# Autodesk Inventor assembly: TTB Constant Force Spring Mount
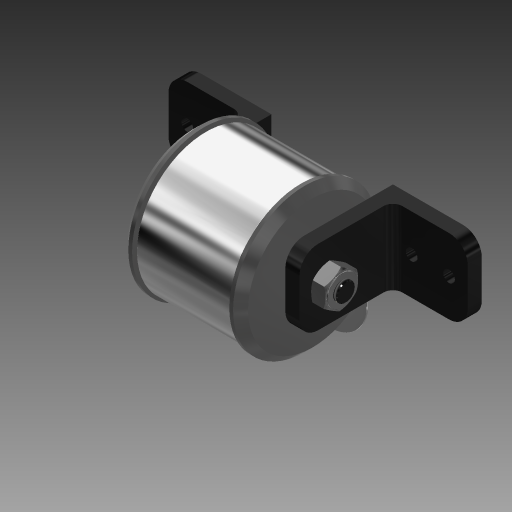
[picture p0: Inventor's stored thumbnail of the model, 512x512]
Saved by Autodesk Inventor 2023 (Build 270158000, 158)
## iProperties
Created: 2023-01-02
Part Number: TTB Constant Force Spring Mount
Document SubType Name: Assembly
Designer: Max Boord
Mass: 227.424 g
Surface Area: 355.542 cm^2
Volume: 75.7539 cm^3
Density: 3.00214 g/cm^3
Author: Max Boord
## iProperties of the stored document MemberDocs/xLcoxz3ngAkn1iylbNymdpbul3h
Created: 2023-01-02
Part Number: TTB Constant Force Spring Mount
Document SubType Name: Assembly
Designer: Max Boord
Mass: 227.424 g
Surface Area: 355.542 cm^2
Volume: 75.7539 cm^3
Density: 3.00214 g/cm^3
Author: Max Boord
## iProperties of the stored document MemberDocs/xGhi35hn1CcuvibzmIsh5smhaFd
Created: 2023-01-02
Part Number: TTB Constant Force Spring Mount
Document SubType Name: Assembly
Designer: Max Boord
Mass: 227.424 g
Surface Area: 355.542 cm^2
Volume: 75.7539 cm^3
Density: 3.00214 g/cm^3
Author: Max Boord
## Documents named in this file (9)
- E:\Collaborative Robots\Collaborative Part Library\Elevators\ThriftyBot Elevator Parts\TTB Constant Force Spring Mount.iam
- E:\Collaborative Robots\Collaborative Part Library\Elevators\ThriftyBot Elevator Parts\TTB Constant Force Spring Spool (ELEV-SPRING-003).ipt
- E:\Collaborative Robots\Collaborative Part Library\Elevators\ThriftyBot Elevator Parts\TTB Constant Force Spring Retainer (ELEV-SPRING-004).ipt
- E:\Collaborative Robots\Collaborative Part Library\Elevators\ThriftyBot Elevator Parts\TTB Constant Force Spring Bracket (ELEV-SPRING-001).ipt
- E:\Collaborative Robots\Collaborative Part Library\Elevators\ThriftyBot Elevator Parts\TTB Elevator Constant Force Spring.ipt
- E:\Collaborative Robots\Collaborative Part Library\Hardware\Fasteners\Machine Screws.ipt
- E:\Collaborative Robots\Collaborative Part Library\Hardware\Fasteners\Machine Screws\1(_FS)4-20 UNCx2.25 Socket Head Cap Screw.ipt
- E:\Collaborative Robots\Collaborative Part Library\Hardware\Nuts and Threaded Blocks\Nuts\1(_FS)4(_DQ)-20 Pan Head Nylon locknut.ipt
- E:\Collaborative Robots\Collaborative Part Library\Hardware\Nuts and Threaded Blocks\Nuts.ipt
## Components (8 placed, 6 different names)
1. TTB Constant Force Spring Spool (ELEV-SPRING-003):1 — Insert:1, Insert:2, Mate:3
2. TTB Constant Force Spring Retainer (ELEV-SPRING-004):1 — Insert:2, Symmetry:3
3. TTB Constant Force Spring Bracket (ELEV-SPRING-001):1 — Flush:1, Mate:1, Mate:2, Mate:3, Symmetry:4, Insert:3, Angle:2, Symmetry:5, Symmetry:6, Tangent:1
4. TTB Constant Force Spring Retainer (ELEV-SPRING-004):2 — Insert:1, Symmetry:3
5. TTB Constant Force Spring Bracket (ELEV-SPRING-001):2 — Flush:1, Mate:1, Mate:2, Angle:1, Symmetry:4, Insert:4, Mate:5, Symmetry:5, Symmetry:6
6. TTB Elevator Constant Force Spring:1 — Angle:1, Mate:6, Flush:2, Tangent:1
7. 1(_FS)4-20 UNCx2.25 Socket Head Cap Screw:1 — Insert:3
8. 1(_FS)4(_DQ)-20 Pan Head Nylon locknut:1 — Insert:4
## Relationships (18: Mate 5, Insert 4, Symmetry 4, Flush 2, Angle 2, Tangent 1)
- Insert:1: TTB Constant Force Spring Spool (ELEV-SPRING-003):1 ↔ TTB Constant Force Spring Retainer (ELEV-SPRING-004):2
- Insert:2: TTB Constant Force Spring Spool (ELEV-SPRING-003):1 ↔ TTB Constant Force Spring Retainer (ELEV-SPRING-004):1
- Flush:1: TTB Constant Force Spring Bracket (ELEV-SPRING-001):1 ↔ TTB Constant Force Spring Bracket (ELEV-SPRING-001):2
- Mate:1: TTB Constant Force Spring Bracket (ELEV-SPRING-001):1 ↔ TTB Constant Force Spring Bracket (ELEV-SPRING-001):2
- Mate:2 (41.2496 mm): TTB Constant Force Spring Bracket (ELEV-SPRING-001):1 ↔ TTB Constant Force Spring Bracket (ELEV-SPRING-001):2
- Mate:3: TTB Constant Force Spring Spool (ELEV-SPRING-003):1 ↔ TTB Constant Force Spring Bracket (ELEV-SPRING-001):1
- Angle:1 (0 deg): TTB Constant Force Spring Bracket (ELEV-SPRING-001):2 ↔ TTB Elevator Constant Force Spring:1
- Symmetry:3: TTB Constant Force Spring Retainer (ELEV-SPRING-004):1 ↔ TTB Constant Force Spring Retainer (ELEV-SPRING-004):2
- Symmetry:4: TTB Constant Force Spring Bracket (ELEV-SPRING-001):1 ↔ TTB Constant Force Spring Bracket (ELEV-SPRING-001):2
- Insert:3: TTB Constant Force Spring Bracket (ELEV-SPRING-001):1 ↔ 1(_FS)4-20 UNCx2.25 Socket Head Cap Screw:1
- Insert:4: TTB Constant Force Spring Bracket (ELEV-SPRING-001):2 ↔ 1(_FS)4(_DQ)-20 Pan Head Nylon locknut:1
- Mate:5: TTB Constant Force Spring Bracket (ELEV-SPRING-001):2
- Angle:2 (0 deg): TTB Constant Force Spring Bracket (ELEV-SPRING-001):1
- Symmetry:5: TTB Constant Force Spring Bracket (ELEV-SPRING-001):1 ↔ TTB Constant Force Spring Bracket (ELEV-SPRING-001):2
- Symmetry:6: TTB Constant Force Spring Bracket (ELEV-SPRING-001):1 ↔ TTB Constant Force Spring Bracket (ELEV-SPRING-001):2
- Mate:6: TTB Elevator Constant Force Spring:1
- Flush:2: TTB Elevator Constant Force Spring:1
- Tangent:1 (-3.3655 mm): TTB Constant Force Spring Bracket (ELEV-SPRING-001):1 ↔ TTB Elevator Constant Force Spring:1
